# Autodesk Inventor assembly: b3
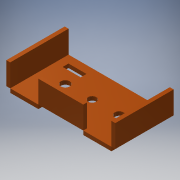
[picture p0: Inventor's stored thumbnail of the model, 180x180]
Saved by Autodesk Inventor 2017 (Build 210142000, 142)
## iProperties
Created: 2016-06-11
Part Number: b3
Document SubType Name: Assembly
Designer: daniel
Author: daniel
## Documents named in this file (4)
- C:\Users\daniel\Documents\GitHub\cardboard-stage-metric\stage\b3.iam
- C:\Users\daniel\Documents\GitHub\cardboard-stage-metric\stage\b3a.ipt
- C:\Users\daniel\Documents\GitHub\cardboard-stage-metric\stage\b3b.ipt
- C:\Users\daniel\Documents\GitHub\cardboard-stage-metric\stage\b3c.ipt
## Components (4 placed, 3 different names)
1. b3a:1 — Mate:1, Mate:2, Mate:3, Mate:4, Mate:5, Flush:1, Flush:2, Mate:6, Mate:7, Mate:8, Mate:9, Mate:10, Mate:11, Flush:3
2. b3b:1 — Mate:4, Mate:5, Flush:1, Mate:8, Mate:10, Flush:3, Flush:4
3. b3c:1 — Mate:1, Mate:2, Mate:3
4. b3b:2 — Flush:2, Mate:6, Mate:7, Mate:9, Mate:11, Flush:4
## Relationships (15: Mate 11, Flush 4)
- Mate:1: b3a:1 ↔ b3c:1
- Mate:2: b3a:1 ↔ b3c:1
- Mate:3: b3a:1 ↔ b3c:1
- Mate:4: b3a:1 ↔ b3b:1
- Mate:5: b3a:1 ↔ b3b:1
- Flush:1: b3a:1 ↔ b3b:1
- Flush:2: b3a:1 ↔ b3b:2
- Mate:6: b3a:1 ↔ b3b:2
- Mate:7: b3a:1 ↔ b3b:2
- Mate:8: b3a:1 ↔ b3b:1
- Mate:9: b3a:1 ↔ b3b:2
- Mate:10: b3a:1 ↔ b3b:1
- Mate:11: b3a:1 ↔ b3b:2
- Flush:3: b3a:1 ↔ b3b:1
- Flush:4: b3b:1 ↔ b3b:2
